# Autodesk Inventor assembly: Caster Wheel
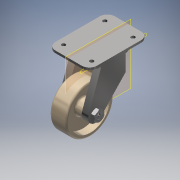
[picture p0: Inventor's stored thumbnail of the model, 180x180]
Saved by Autodesk Inventor 2017 (Build 210142000, 142)
## iProperties
Created: 2016-06-16
Part Number: Caster Wheel
Document SubType Name: Assembly
Designer: Dakota Marin
Author: Dakota Marin
## Documents named in this file (5)
- C:\Users\Dakota Marin\Desktop\CAD Projects\Caster Wheel Type 1\Caster Wheel.iam
- C:\Users\Dakota Marin\Desktop\CAD Projects\Caster Wheel Type 1\Plate2.ipt
- C:\Users\Dakota Marin\Desktop\CAD Projects\Caster Wheel Type 1\Wheel.ipt
- C:\Users\Dakota Marin\Desktop\CAD Projects\Caster Wheel Type 1\Nut.ipt
- C:\Users\Dakota Marin\Desktop\CAD Projects\Caster Wheel Type 1\Thread.ipt
## Components (5 placed, 4 different names)
1. Plate2:1 — Mate:1, Mate:2, Mate:3
2. Wheel:1
3. Nut:1 — Mate:3
4. Thread:1 — Mate:2
5. Nut:2 — Mate:1
## Relationships (3: Mate 3)
- Mate:1: Plate2:1 ↔ Nut:2
- Mate:2: Plate2:1 ↔ Thread:1
- Mate:3: Plate2:1 ↔ Nut:1
